# Autodesk Inventor assembly: Assembly_Z_stage
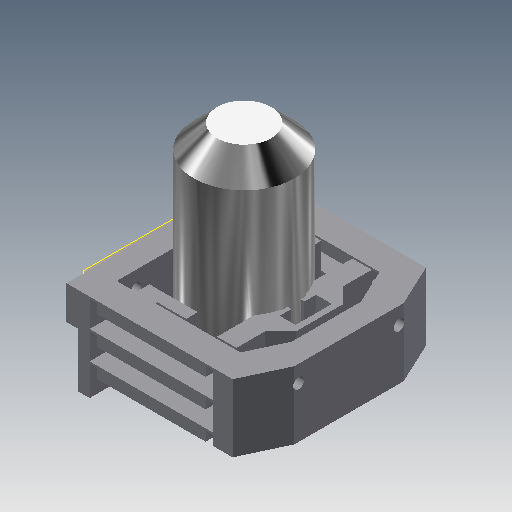
[picture p0: Inventor's stored thumbnail of the model, 512x512]
Saved by Autodesk Inventor 2019 (Build 230136000, 136)
## iProperties
Created: 2020-04-29
Part Number: Assembly_Z_stage
Document SubType Name: Assembly
Designer: diederichbenedict
Author: diederichbenedict
## Documents named in this file (4)
- C:\Users\diederichbenedict\Dropbox\Dokumente\Promotion\PROJECTS\STORMoChip\GITHUB\CAD\Nanoscopy-on-the-cheap\Workspace\Assembly_Z_stage.iam
- C:\Users\diederichbenedict\Dropbox\Dokumente\Promotion\PROJECTS\STORMoChip\GITHUB\CAD\Nanoscopy-on-the-cheap\Workspace\cellSTORM_v5_focussingunit_1.ipt
- C:\Users\diederichbenedict\Dropbox\Dokumente\Promotion\PROJECTS\STORMoChip\GITHUB\CAD\Nanoscopy-on-the-cheap\Workspace\cellSTORM_objective_thread.ipt
- C:\Users\diederichbenedict\Dropbox\Dokumente\Promotion\PROJECTS\STORMoChip\GITHUB\CAD\Nanoscopy-on-the-cheap\Workspace\00_Microscope_Objective.ipt
## Components (3 placed, 3 different names)
1. cellSTORM_v5_focussingunit_1:1 — Mate:1, Angle:1, Angle:2
2. cellSTORM_objective_thread:1 — Mate:1, Angle:1, Insert:1
3. 00_Microscope_Objective:1 — Insert:1, Angle:2
## Relationships (4: Angle 2, Mate 1, Insert 1)
- Mate:1: cellSTORM_v5_focussingunit_1:1 ↔ cellSTORM_objective_thread:1
- Angle:1 (0 deg): cellSTORM_v5_focussingunit_1:1 ↔ cellSTORM_objective_thread:1
- Insert:1: cellSTORM_objective_thread:1 ↔ 00_Microscope_Objective:1
- Angle:2 (0 deg): cellSTORM_v5_focussingunit_1:1 ↔ 00_Microscope_Objective:1
